# Autodesk Inventor assembly: SteelM-StarS
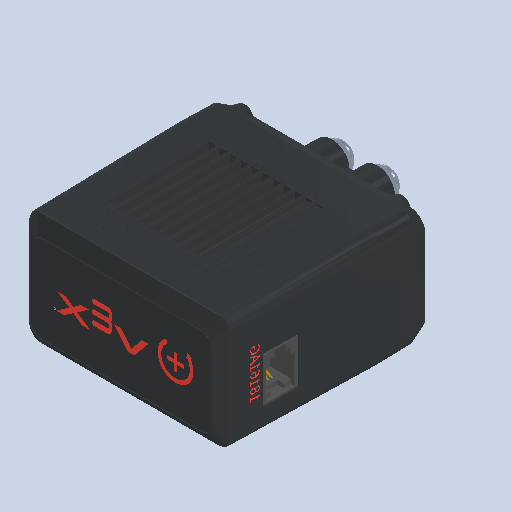
[picture p0: Inventor's stored thumbnail of the model, 512x512]
Saved by Autodesk Inventor 2025.2 (Build 292293000, 293)
## iProperties
Created: 2022-08-18
Part Number: SteelM-StarS
Document SubType Name: Assembly
Designer: avere
Author: ylu12
## Documents named in this file (4)
- D:\vex\cad\v5\Drivetrain\Drivebay Right\SteelM-StarS.iam
- D:\vex\cad\v5\Drivetrain\Drivebay Right\V5 Motor.ipt
- D:\vex\cad\VEX-CAD-Inventor\Structure\Hardware\Screw Steel - Star\SScrew Star Smooth .500.ipt
- D:\vex\cad\VEX-CAD-Inventor\Structure\Hardware\Screw Steel - Star.ipt
## Components (3 placed, 2 different names)
1. V5 Motor:1
2. SScrew Star Smooth .500:1
3. SScrew Star Smooth .500:2
## Named parameters: Thickness = 1.1938 mm
